# Autodesk Inventor assembly: Y_Slider_mit_Schrittmorotr
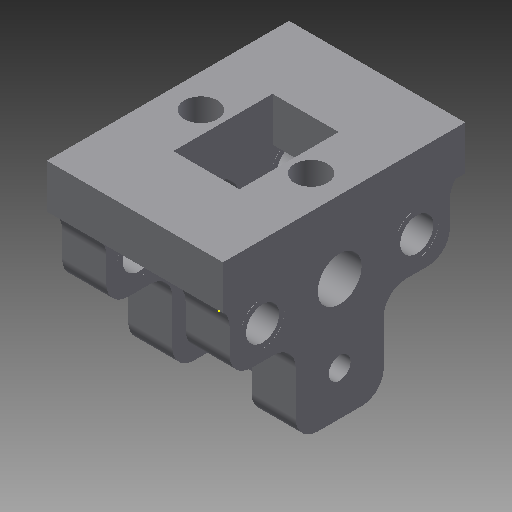
[picture p0: Inventor's stored thumbnail of the model, 512x512]
Saved by Autodesk Inventor 2019 (Build 230136000, 136)
## iProperties
Created: 2018-08-19
Part Number: Y_Slider_mit_Schrittmorotr
Document SubType Name: Assembly
Designer: Julia
Author: Julia
## Documents named in this file (5)
- C:\Users\Julia\Documents\Inventor\3d_Drucker_v02\Y_Slider_mit_Schrittmotor.iam
- C:\Users\Julia\Documents\Inventor\3d_Drucker_v02\Metallstange_Slider.ipt
- C:\Users\Julia\Documents\Inventor\3d_Drucker_v02\Y_Slider_Zahnrad_Stange.ipt
- C:\Users\Julia\Documents\Inventor\3d_Drucker_v02\Y_Slider_Zahnrad.ipt
- C:\Users\Julia\Documents\Inventor\3d_Drucker_v02\Y_Slider_Part_mit_Schrittmotor.ipt
## Components (7 placed, 4 different names)
1. Y_Slider_Part_mit_Schrittmotor:1 — Mate:1, Mate:2, Mate:3, Mate:4, Flush:1, Flush:2, Flush:3, Flush:4, Mate:5, Flush:5, Mate:7
2. Metallstange_Slider:1 — Mate:3, Flush:2
3. Metallstange_Slider:2 — Mate:1, Flush:3
4. Metallstange_Slider:3 — Mate:4, Flush:4
5. Metallstange_Slider:4 — Mate:2, Flush:1
6. Y_Slider_Zahnrad_Stange:1 — Mate:5, Flush:5, Mate:6
7. Y_Slider_Zahnrad:1 — Mate:6, Mate:7
## Relationships (12: Mate 7, Flush 5)
- Mate:1: Y_Slider_Part_mit_Schrittmotor:1 ↔ Metallstange_Slider:2
- Mate:2: Y_Slider_Part_mit_Schrittmotor:1 ↔ Metallstange_Slider:4
- Mate:3: Y_Slider_Part_mit_Schrittmotor:1 ↔ Metallstange_Slider:1
- Mate:4: Y_Slider_Part_mit_Schrittmotor:1 ↔ Metallstange_Slider:3
- Flush:1: Y_Slider_Part_mit_Schrittmotor:1 ↔ Metallstange_Slider:4
- Flush:2: Y_Slider_Part_mit_Schrittmotor:1 ↔ Metallstange_Slider:1
- Flush:3: Y_Slider_Part_mit_Schrittmotor:1 ↔ Metallstange_Slider:2
- Flush:4: Y_Slider_Part_mit_Schrittmotor:1 ↔ Metallstange_Slider:3
- Mate:5: Y_Slider_Part_mit_Schrittmotor:1 ↔ Y_Slider_Zahnrad_Stange:1
- Flush:5: Y_Slider_Part_mit_Schrittmotor:1 ↔ Y_Slider_Zahnrad_Stange:1
- Mate:6: Y_Slider_Zahnrad_Stange:1 ↔ Y_Slider_Zahnrad:1
- Mate:7 (10.5 mm): Y_Slider_Part_mit_Schrittmotor:1 ↔ Y_Slider_Zahnrad:1
